# Autodesk Inventor assembly: PoweredWheelAssembly_MIR
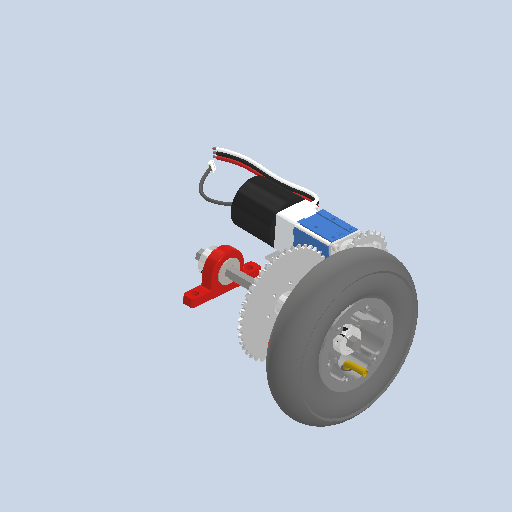
[picture p0: Inventor's stored thumbnail of the model, 512x512]
Saved by Autodesk Inventor 2023 (Build 270158000, 158)
## iProperties
Created: 2022-09-14
Part Number: PoweredWheelAssembly_MIR
Document SubType Name: Assembly
Designer: PC
Author: PC
## Documents named in this file (12)
- C:\Users\PC\Documents\PersonalCAD\ARCIGVC\IGVC-Robot\PoweredWheelAssembly_MIR.iam
- C:\Users\PC\Documents\PersonalCAD\ARCIGVC\IGVC-Robot\8inPneumatic_MIR.ipt
- C:\Users\PC\Documents\PersonalCAD\ARCIGVC\IGVC-Robot\2 Stage HD - CIM Sport_MIR.ipt
- C:\Users\PC\Documents\PersonalCAD\ARCIGVC\IGVC-Robot\am-4258 NEO Brushless Motor_MIR.ipt
- C:\Users\PC\Documents\PersonalCAD\ARCIGVC\IGVC-Robot\MotorMount_MIR.ipt
- C:\Users\PC\Documents\PersonalCAD\ARCIGVC\IGVC-Robot\24tSprocket35Series_MIR.ipt
- C:\Users\PC\Documents\PersonalCAD\ARCIGVC\IGVC-Robot\42tSprocket35Series_MIR.ipt
- C:\Users\PC\Documents\PersonalCAD\ARCIGVC\IGVC-Robot\Hex Hub .5In_MIR.ipt
- C:\Users\PC\Documents\PersonalCAD\ARCIGVC\IGVC-Robot\Bearing Housing_MIR1.ipt
- C:\Users\PC\Documents\PersonalCAD\ARCIGVC\IGVC-Robot\HalfInHex Bearing_MIR.ipt
- C:\Users\PC\Documents\PersonalCAD\ARCIGVC\IGVC-Robot\9in-0.5inHexAxel_MIR.ipt
- C:\Users\PC\Documents\PersonalCAD\ARCIGVC\IGVC-Robot\am-1526 500Hex HD Collar Clamp_MIR.ipt
## Components (17 placed, 11 different names)
1. 8inPneumatic_MIR:1 — Mate:35, Mate:23, Mate:27, Flush:3, Mate:34
2. 2 Stage HD - CIM Sport_MIR:1 — Mate:3, Mate:2, Mate:1, Mate:6, Mate:5, Mate:4, Flush:1, Mate:10
3. am-4258 NEO Brushless Motor_MIR:1 — Mate:3, Mate:2, Mate:1
4. MotorMount_MIR:1 — Mate:6, Mate:5, Mate:4, Flush:7, Flush:6, Mate:30
5. 24tSprocket35Series_MIR:1 — Flush:2, Mate:9, Mate:8, Mate:7
6. 42tSprocket35Series_MIR:1 — Flush:2, Mate:13, Mate:12, Mate:11
7. Hex Hub .5In_MIR:1 — Mate:13, Mate:12, Mate:11, Mate:24, Mate:26, Mate:25
8. Hex Hub .5In_MIR:2 — Flush:1, Mate:10, Mate:9, Mate:8, Mate:7
9. Bearing Housing_MIR1:1 — Mate:35, Mate:24, Mate:23, Flush:4, Mate:14, Mate:16, Mate:15, Mate:18, Mate:17
10. Bearing Housing_MIR1:2 — Flush:7, Flush:6, Flush:4, Mate:14, Mate:30, Mate:22, Mate:19, Mate:21, Mate:20, Flush:5
11. HalfInHex Bearing_MIR:1 — Mate:16, Mate:15
12. HalfInHex Bearing_MIR:2 — Mate:18, Mate:17
13. HalfInHex Bearing_MIR:3 — Mate:22, Mate:19, Mate:31
14. HalfInHex Bearing_MIR:4 — Mate:21, Mate:20
15. 9in-0.5inHexAxel_MIR:1 — Flush:5, Mate:27, Flush:3, Mate:26, Mate:25, Mate:33, Mate:32, Mate:29, Mate:28
16. am-1526 500Hex HD Collar Clamp_MIR:1 — Mate:34, Mate:33, Mate:32
17. am-1526 500Hex HD Collar Clamp_MIR:2 — Mate:31, Mate:29, Mate:28
## Relationships (42: Mate 35, Flush 7)
- Mate:3: 2 Stage HD - CIM Sport_MIR:1 ↔ am-4258 NEO Brushless Motor_MIR:1
- Mate:2: 2 Stage HD - CIM Sport_MIR:1 ↔ am-4258 NEO Brushless Motor_MIR:1
- Mate:1: 2 Stage HD - CIM Sport_MIR:1 ↔ am-4258 NEO Brushless Motor_MIR:1
- Mate:6: 2 Stage HD - CIM Sport_MIR:1 ↔ MotorMount_MIR:1
- Mate:5: 2 Stage HD - CIM Sport_MIR:1 ↔ MotorMount_MIR:1
- Mate:4: 2 Stage HD - CIM Sport_MIR:1 ↔ MotorMount_MIR:1
- Flush:2: 24tSprocket35Series_MIR:1 ↔ 42tSprocket35Series_MIR:1
- Mate:13: 42tSprocket35Series_MIR:1 ↔ Hex Hub .5In_MIR:1
- Mate:12: 42tSprocket35Series_MIR:1 ↔ Hex Hub .5In_MIR:1
- Mate:11: 42tSprocket35Series_MIR:1 ↔ Hex Hub .5In_MIR:1
- Flush:1: 2 Stage HD - CIM Sport_MIR:1 ↔ Hex Hub .5In_MIR:2
- Mate:10: 2 Stage HD - CIM Sport_MIR:1 ↔ Hex Hub .5In_MIR:2
- Mate:9: 24tSprocket35Series_MIR:1 ↔ Hex Hub .5In_MIR:2
- Mate:8: 24tSprocket35Series_MIR:1 ↔ Hex Hub .5In_MIR:2
- Mate:7: 24tSprocket35Series_MIR:1 ↔ Hex Hub .5In_MIR:2
- Mate:35 (17.4752 mm): 8inPneumatic_MIR:1 ↔ Bearing Housing_MIR1:1
- Mate:24: Hex Hub .5In_MIR:1 ↔ Bearing Housing_MIR1:1
- Mate:23: 8inPneumatic_MIR:1 ↔ Bearing Housing_MIR1:1
- Flush:7: MotorMount_MIR:1 ↔ Bearing Housing_MIR1:2
- Flush:6 (4.7752 mm): MotorMount_MIR:1 ↔ Bearing Housing_MIR1:2
- Flush:4: Bearing Housing_MIR1:1 ↔ Bearing Housing_MIR1:2
- Mate:14: Bearing Housing_MIR1:1 ↔ Bearing Housing_MIR1:2
- Mate:30 (25.4 mm): MotorMount_MIR:1 ↔ Bearing Housing_MIR1:2
- Mate:16: Bearing Housing_MIR1:1 ↔ HalfInHex Bearing_MIR:1
- Mate:15: Bearing Housing_MIR1:1 ↔ HalfInHex Bearing_MIR:1
- Mate:18: Bearing Housing_MIR1:1 ↔ HalfInHex Bearing_MIR:2
- Mate:17: Bearing Housing_MIR1:1 ↔ HalfInHex Bearing_MIR:2
- Mate:22: Bearing Housing_MIR1:2 ↔ HalfInHex Bearing_MIR:3
- Mate:19: Bearing Housing_MIR1:2 ↔ HalfInHex Bearing_MIR:3
- Mate:21: Bearing Housing_MIR1:2 ↔ HalfInHex Bearing_MIR:4
- Mate:20: Bearing Housing_MIR1:2 ↔ HalfInHex Bearing_MIR:4
- Flush:5 (25.5778 mm): Bearing Housing_MIR1:2 ↔ 9in-0.5inHexAxel_MIR:1
- Mate:27: 8inPneumatic_MIR:1 ↔ 9in-0.5inHexAxel_MIR:1
- Flush:3: 8inPneumatic_MIR:1 ↔ 9in-0.5inHexAxel_MIR:1
- Mate:26: Hex Hub .5In_MIR:1 ↔ 9in-0.5inHexAxel_MIR:1
- Mate:25: Hex Hub .5In_MIR:1 ↔ 9in-0.5inHexAxel_MIR:1
- Mate:34: 8inPneumatic_MIR:1 ↔ am-1526 500Hex HD Collar Clamp_MIR:1
- Mate:33: 9in-0.5inHexAxel_MIR:1 ↔ am-1526 500Hex HD Collar Clamp_MIR:1
- Mate:32: 9in-0.5inHexAxel_MIR:1 ↔ am-1526 500Hex HD Collar Clamp_MIR:1
- Mate:31: HalfInHex Bearing_MIR:3 ↔ am-1526 500Hex HD Collar Clamp_MIR:2
- Mate:29: 9in-0.5inHexAxel_MIR:1 ↔ am-1526 500Hex HD Collar Clamp_MIR:2
- Mate:28: 9in-0.5inHexAxel_MIR:1 ↔ am-1526 500Hex HD Collar Clamp_MIR:2
